# Autodesk Inventor assembly: HBLBS5
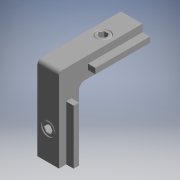
[picture p0: Inventor's stored thumbnail of the model, 180x180]
Saved by Autodesk Inventor 2017.3 (Build 213256000, 256)
## iProperties
Category: PARTsolutions
Company: MISUMI
Part Number: HBLBS5
Catalog Web Link: www.cadenas.de
Description: HBLBS5, SHBLBS5-Brackets HFS5 Blind Brackets
Vendor: MISUMI
Document SubType Name: Assembly
Designer: partserver
Manufacturer: MISUMI
Mass: 1.51453 g
Surface Area: 15.0258 cm^2
Volume: 1.51453 cm^3
Density: 1 g/cm^3
Title: HBLBS5
Author: Cadenas PARTsolutions
Comments: Brackets HFS5 Blind Brackets
PSOL_IDENT_0: {$CADENAS_DATA\23d-libs\misumi\metric\38_al_extrusions_blackets\5\shblbs5_asmtab.prj},166 {VTYP=3D},
PSOL_IDENT_1: {STYP=ASSTAB},{NB=HBLBS5},{LINA=HBLBS5},{NN=HBLBS5, SHBLBS5},{DATE=08.06.2021 08:25:23},{GEOMDATE=25
PSOL_IDENT_2: .08.2009},{VERSION=},{LINEID=60},{WBVAR=},{WBNUMERIC=}  {NB=HBLBS5},{LINA=HBLBS5},{KT=1},{PN=HBLBS5}
PSOL_IDENT_3: ,{VERS=1},{MAT=1045 Carbon Steel},{ST=Trivalent Chromate},{MASS=11},{AB=Set Screw M4x5 (Attached)},{
PSOL_IDENT_4: NOB=2},{MATN=-},{MATS=-},{AL=196},{PPATH=hblbs5_asmtpl.prj}
NB: HBLBS5
NN: HBLBS5, SHBLBS5
NT: Brackets HFS5 Blind Brackets
NBSYN: $PN.
LINA: HBLBS5
CATALOG: Misumi
PN: HBLBS5
MAT: 1045 Carbon Steel
ST: Trivalent Chromate Plating
MASS: 11
AB: Set Screw M4x5 (Attached)
NOB: 2
AL: 196
SUPPLIER: MISUMI
ARTICLENO: HBLBS5
BOMINFO: HBLBS5
CREATOR: CADENAS GmbH
## Documents named in this file (3)
- e:\temp\worker_2\temp\exporttempdir_4460_34_jJW25\format_0\HBLBS5.iam
- e:\temp\worker_2\temp\exporttempdir_4460_34_jJW25\format_0\HBLBS5b.ipt
- e:\temp\worker_2\temp\exporttempdir_4460_34_jJW25\format_0\Hexagon socket set screw with flat point DIN 913 - M4x5.ipt
## Components (3 placed, 2 different names)
1. HBLBS5b:1 — bracket_to_screw1_Z@1 <-> IP2_Z@2, bracket_to_screw2_Z@1 <-> IP2_Z@3
2. Hexagon socket set screw with flat point DIN 913 - M4x5:1 — bracket_to_screw1_Z@1 <-> IP2_Z@2
3. Hexagon socket set screw with flat point DIN 913 - M4x5:2 — bracket_to_screw2_Z@1 <-> IP2_Z@3
## Relationships (2: Mate 2)
- bracket_to_screw1_Z@1 <-> IP2_Z@2 [Mate]: HBLBS5b:1 ↔ Hexagon socket set screw with flat point DIN 913 - M4x5:1
- bracket_to_screw2_Z@1 <-> IP2_Z@3 [Mate]: HBLBS5b:1 ↔ Hexagon socket set screw with flat point DIN 913 - M4x5:2
